# Autodesk Inventor assembly: Manipulator_Sterowniki_Robotów
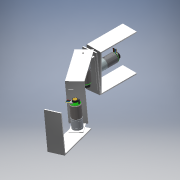
[picture p0: Inventor's stored thumbnail of the model, 180x180]
Saved by Autodesk Inventor 2019 (Build 230136000, 136)
## iProperties
Created: 2021-05-21
Part Number: Manipulator_Sterowniki_Robotów
Document SubType Name: Assembly
Designer: DOMEK
Sending System: SIEMENS PLM Software NX 1907
Preprocessor: ST-DEVELOPER v16.7
Title: Manipulator_Sterowniki_Robotów.stp
## Documents named in this file (8)
- D:\Manipulator\Inventor-20\Manipulator_Sterowniki_Robotów.iam
- D:\Manipulator\Inventor-20\Manipulator_Pierwszy_Stopien.ipt
- D:\Manipulator\Inventor-20\25d-metal-gearmotor-172-227-encoder_step.ipt
- D:\Manipulator\Inventor-20\Manipulator_DolnyHolderSilnika.ipt
- D:\Manipulator\Inventor-20\Manipulator_Handler_Silnikow.ipt
- D:\Manipulator\Inventor-20\25d-metal-gearmotor-172-227-encoder.ipt
- D:\Manipulator\Inventor-20\Manipulator_DrugiStopien.ipt
- D:\Manipulator\Inventor-20\Manipulator_TrzeciStopien.ipt
## Components (9 placed, 7 different names)
1. Manipulator_Pierwszy_Stopien_1002
2. 25d-metal-gearmotor-172-227-encoder_step_1003 — Insert:1, Insert:2
3. Manipulator_DolnyHolderSilnika:1 — Insert:1, Flush:4
4. Manipulator_Handler_Silnikow:1 — Insert:2, Insert:4, Insert:5, Flush:4
5. 25d-metal-gearmotor-172-227-encoder:1 — Insert:4, Insert:5, Insert:6
6. Manipulator_DrugiStopien:1 — Insert:6, Mate:1, Flush:1, Flush:5
7. Manipulator_Handler_Silnikow:2 — Mate:1, Flush:1, Insert:7, Insert:8, Flush:5
8. 25d-metal-gearmotor-172-227-encoder:2 — Insert:7, Insert:8, Insert:9
9. Manipulator_TrzeciStopien:1 — Insert:9
## Relationships (12: Insert 8, Flush 3, Mate 1)
- Insert:1 (-5 mm): 25d-metal-gearmotor-172-227-encoder_step_1003 ↔ Manipulator_DolnyHolderSilnika:1
- Insert:2 (-2 mm): 25d-metal-gearmotor-172-227-encoder_step_1003 ↔ Manipulator_Handler_Silnikow:1
- Insert:4: Manipulator_Handler_Silnikow:1 ↔ 25d-metal-gearmotor-172-227-encoder:1
- Insert:5: Manipulator_Handler_Silnikow:1 ↔ 25d-metal-gearmotor-172-227-encoder:1
- Insert:6 (-4 mm): 25d-metal-gearmotor-172-227-encoder:1 ↔ Manipulator_DrugiStopien:1
- Mate:1: Manipulator_DrugiStopien:1 ↔ Manipulator_Handler_Silnikow:2
- Flush:1: Manipulator_DrugiStopien:1 ↔ Manipulator_Handler_Silnikow:2
- Insert:7: Manipulator_Handler_Silnikow:2 ↔ 25d-metal-gearmotor-172-227-encoder:2
- Insert:8: Manipulator_Handler_Silnikow:2 ↔ 25d-metal-gearmotor-172-227-encoder:2
- Flush:4 (2 mm): Manipulator_DolnyHolderSilnika:1 ↔ Manipulator_Handler_Silnikow:1
- Flush:5 (4 mm): Manipulator_DrugiStopien:1 ↔ Manipulator_Handler_Silnikow:2
- Insert:9 (-4 mm): 25d-metal-gearmotor-172-227-encoder:2 ↔ Manipulator_TrzeciStopien:1
